# Autodesk Inventor assembly: main climber
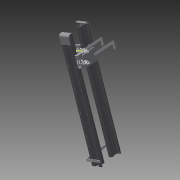
[picture p0: Inventor's stored thumbnail of the model, 180x180]
Saved by Autodesk Inventor 2013 (Build 170138000, 138)
## iProperties
Created: 2013-01-25
Part Number: main climber
Document SubType Name: Assembly
Designer: Arpan
Author: Arpan
## Documents named in this file (8)
- C:\Users\Arpan\Documents\GitHub\frc2013CAD\Cimber actual\main climber.iam
- C:\Users\Arpan\Documents\GitHub\frc2013CAD\Cimber actual\Shaft 26 inch.ipt
- C:\Users\Arpan\Documents\GitHub\frc2013CAD\Cimber actual\Bearing Block long style.iam
- C:\Users\Arpan\Documents\GitHub\frc2013CAD\Cimber actual\hook mount plate.ipt
- C:\Users\Arpan\Documents\GitHub\frc2013CAD\Cimber actual\tie-together tier 1.ipt
- C:\Users\Arpan\Documents\GitHub\frc2013CAD\Cimber actual\endstop.ipt
- C:\Users\Arpan\Documents\GitHub\frc2013CAD\Cimber actual\hook faceplate.ipt
- C:\Users\Arpan\Documents\GitHub\frc2013CAD\Cimber actual\hook.ipt
## Components (12 placed, 7 different names)
1. Shaft 26 inch:1 — Flush:1, Angle:1, Mate:2, Flush:2, Angle:2, Mate:12, Mate:13, Flush:8
2. Shaft 26 inch:2 — Flush:1, Angle:1, Mate:1, Flush:2, Mate:7, Mate:8, Mate:9, Flush:7, Mate:10, Mate:11
3. Bearing Block long style:1 [sub-assembly] — Mate:1, Mate:3, Flush:3, Mate:16, Mate:17
4. Bearing Block long style:2 [sub-assembly] — Mate:2, Mate:3, Angle:2, Flush:3, Mate:14, Flush:9, Mate:15
5. hook mount plate:1 — Mate:14, Flush:9, Mate:15, Flush:10, Mate:18, Flush:11, Flush:12
6. hook mount plate:2 — Mate:16, Mate:17, Flush:10
7. tie-together tier 1:1 — Mate:7, Mate:8, Mate:9
8. endstop:1 — Mate:12, Mate:13, Flush:8
9. endstop:2 — Flush:7, Mate:10, Mate:11
10. hook faceplate:1 — Mate:18, Flush:11, Flush:12, Mate:19, Mate:20, Mate:21, Mate:22, Flush:13, Flush:14
11. hook:1 — Mate:19, Mate:22, Flush:14
12. hook:2 — Mate:20, Mate:21, Flush:13
## Relationships (32: Mate 19, Flush 11, Angle 2)
- Flush:1: Shaft 26 inch:1 ↔ Shaft 26 inch:2
- Angle:1 (180 deg): Shaft 26 inch:1 ↔ Shaft 26 inch:2
- Mate:1: Shaft 26 inch:2 ↔ Bearing Block long style:1
- Mate:2: Shaft 26 inch:1 ↔ Bearing Block long style:2
- Mate:3 (12.7 mm): Bearing Block long style:1 ↔ Bearing Block long style:2
- Flush:2: Shaft 26 inch:1 ↔ Shaft 26 inch:2
- Angle:2 (0 deg): Shaft 26 inch:1 ↔ Bearing Block long style:2
- Flush:3: Bearing Block long style:1 ↔ Bearing Block long style:2
- Mate:7 (25.4 mm): Shaft 26 inch:2 ↔ tie-together tier 1:1
- Mate:8: Shaft 26 inch:2 ↔ tie-together tier 1:1
- Mate:9 (23.4188 mm): Shaft 26 inch:2 ↔ tie-together tier 1:1
- Flush:7: Shaft 26 inch:2 ↔ endstop:2
- Mate:10: Shaft 26 inch:2 ↔ endstop:2
- Mate:11: Shaft 26 inch:2 ↔ endstop:2
- Mate:12: Shaft 26 inch:1 ↔ endstop:1
- Mate:13: Shaft 26 inch:1 ↔ endstop:1
- Flush:8: Shaft 26 inch:1 ↔ endstop:1
- Mate:14: Bearing Block long style:2 ↔ hook mount plate:1
- Flush:9: Bearing Block long style:2 ↔ hook mount plate:1
- Mate:15: Bearing Block long style:2 ↔ hook mount plate:1
- Mate:16: Bearing Block long style:1 ↔ hook mount plate:2
- Mate:17: Bearing Block long style:1 ↔ hook mount plate:2
- Flush:10: hook mount plate:1 ↔ hook mount plate:2
- Mate:18: hook mount plate:1 ↔ hook faceplate:1
- Flush:11: hook mount plate:1 ↔ hook faceplate:1
- Flush:12 (38.1 mm): hook mount plate:1 ↔ hook faceplate:1
- Mate:19: hook faceplate:1 ↔ hook:1
- Mate:20: hook faceplate:1 ↔ hook:2
- Mate:21 (-26.1747 mm): hook faceplate:1 ↔ hook:2
- Mate:22 (26.1874 mm): hook faceplate:1 ↔ hook:1
- Flush:13 (6.35 mm): hook faceplate:1 ↔ hook:2
- Flush:14 (6.35 mm): hook faceplate:1 ↔ hook:1
